# Autodesk Inventor assembly: BSPG15-60 (40)
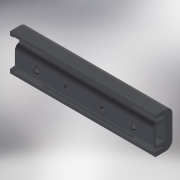
[picture p0: Inventor's stored thumbnail of the model, 180x180]
Saved by Autodesk Inventor 2016 (Build 200138000, 138)
## iProperties
Category: PARTsolutions
Company: IKO
Created: 2015-05-07
Part Number: BSPG15-60 (40)
Catalog Web Link: www.cadenas.de
Description: BSPG-
Vendor: IKO
Document SubType Name: Assembly
Designer: PARTuser1
Manufacturer: IKO
Mass: 3.65172 g
Surface Area: 70.2562 cm^2
Volume: 3.65172 cm^3
Density: 1 g/cm^3
PSOL_IDENT_0: {$CADENAS_DATA\23d-libs\iko\linear_way_series\precise_ball_slide\bspg_asmtab.prj},172 {VTYP=3D},{STY
PSOL_IDENT_1: P=ASSTAB},{NB=BSPG15-60 (40)},{LINA=BSPG15-60},{NN=BSPG},{DATE=18.01.2008 10:02:28},{GEOMDATE=11.10.
PSOL_IDENT_2: 2007},{VERSION=},{LINEID=10},{LINESUBID=-1},{WBVAR=SZ,L}  {NB=BSPG15-60 (40)},{LINA=BSPG15-60},{KT=D
PSOL_IDENT_3: UMMY},{IDNR=},{MN=BSPG},{SZ=15},{L=60},{LX=40,50,60},{MS=40},{PPATH=bspg_asmtpl.prj}
SUPPLIER: IKO
ARTICLENO: BSPG15-60 (40)
BOMINFO: BSPG15-60
CREATOR: CADENAS GmbH
Title: BSPG15-60
Author: Cadenas PARTsolutions
## Documents named in this file (4)
- C:\Users\as\Documents\Inventor\mintplacer-export\BSPG15_60__40_.iam
- C:\Users\as\Documents\Inventor\mintplacer-export\BSPG1560_Table.ipt
- C:\Users\as\Documents\Inventor\mintplacer-export\BSPG_SL1560Retainer.ipt
- C:\Users\as\Documents\Inventor\mintplacer-export\BSPG1560_Rail.ipt
## Components (3 placed, 3 different names)
1. BSPG1560_Table:1 — Flush:1, IKO-T1-slide
2. BSPG_SL1560Retainer:1
3. BSPG1560_Rail:1 — Flush:1, IKO-T1-slide
## Relationships (2: Flush 1, TranslationJoint 1)
- Flush:1 (-2.7 mm): BSPG1560_Table:1 ↔ BSPG1560_Rail:1
- IKO-T1-slide [TranslationJoint] (-8 mm): BSPG1560_Table:1 ↔ BSPG1560_Rail:1
